# Autodesk Inventor assembly: IdleRoller
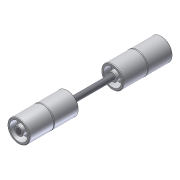
[picture p0: Inventor's stored thumbnail of the model, 180x180]
Saved by Autodesk Inventor 2012 (Build 160160000, 160)
## iProperties
Created: 2012-01-16
Part Number: IdleRoller
Document SubType Name: Assembly
Designer: JesseK
Mass: 207.677 g
Surface Area: 464.881 cm^2
Volume: 100.364 cm^3
Density: 2.06924 g/cm^3
Author: JesseK
## Documents named in this file (3)
- Z:\UserData\Documents\Inventor\team1885frc\Robot2012\Conveyor2\IdleRoller.iam
- Z:\UserData\Documents\Inventor\team1885frc\Robot2012\Conveyor2\RollerAxle.ipt
- Z:\UserData\Documents\Inventor\team1885frc\Robot2012\Conveyor2\Conveyor_Roller_MainOuter.ipt
## Components (5 placed, 2 different names)
1. RollerAxle:1 — Mate:1, Flush:1, Mate:2, Mate:5, Flush:2, Mate:6
2. Conveyor_Roller_MainOuter:1 — Mate:1, Flush:1, Mate:3
3. Conveyor_Roller_MainOuter:2 — Mate:2, Mate:3
4. Conveyor_Roller_MainOuter:4 — Mate:6, Mate:7
5. Conveyor_Roller_MainOuter:5 — Mate:5, Flush:2, Mate:7
## Relationships (8: Mate 6, Flush 2)
- Mate:1: RollerAxle:1 ↔ Conveyor_Roller_MainOuter:1
- Flush:1: RollerAxle:1 ↔ Conveyor_Roller_MainOuter:1
- Mate:2: RollerAxle:1 ↔ Conveyor_Roller_MainOuter:2
- Mate:3: Conveyor_Roller_MainOuter:1 ↔ Conveyor_Roller_MainOuter:2
- Mate:5: RollerAxle:1 ↔ Conveyor_Roller_MainOuter:5
- Flush:2: RollerAxle:1 ↔ Conveyor_Roller_MainOuter:5
- Mate:6: RollerAxle:1 ↔ Conveyor_Roller_MainOuter:4
- Mate:7: Conveyor_Roller_MainOuter:4 ↔ Conveyor_Roller_MainOuter:5
